# Autodesk Inventor assembly: Assembly-jig
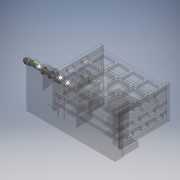
[picture p0: Inventor's stored thumbnail of the model, 180x180]
Saved by Autodesk Inventor 2018 (Build 220112000, 112)
## iProperties
Created: 2017-11-08
Part Number: Assembly-jig
Document SubType Name: Assembly
Designer: xl0
Author: xl0
## Documents named in this file (7)
- E:\Alex\koi\Cuvette-rack\Parts\Assembly-jig\Assembly-jig.iam
- E:\Alex\koi\Cuvette-rack\Parts\Cuvette-rack.iam
- E:\Alex\koi\Cuvette-rack\Parts\Assembly-jig\Assembly-jig-base.ipt
- E:\Alex\koi\Cuvette-rack\Parts\Assembly-jig\Assembly-jig\Design Accelerator\Compress Spring3.iam
- C:\Users\xl0\Documents\Inventor\Content Center Files\R2018\en-US\ANSI B18.2.4.2M\ANSI B18.2.4.2M - M3x0.5 - 5.5.ipt
- C:\Users\xl0\Documents\Inventor\Content Center Files\R2018\en-US\ANSI B18.22 M\ANSI B18.22M - 3 N.ipt
- C:\Users\xl0\Documents\Inventor\Content Center Files\R2018\en-US\SS-ISO 4762\ISO 4762 - M4 x 40SS-ISO.ipt
## Components (8 placed, 6 different names)
1. Cuvette-rack:1 [sub-assembly] — Flush:1, Flush:4
2. Assembly-jig-base:1 — Flush:1, Flush:4, Mate:1, Mate:8, Mate:9
3. SS ISO 4762 M4 x 40:1 — Mate:1, Mate:2, Flush:5, Mate:3, Mate:4, Mate:6, Mate:7, Flush:6
4. Compress Spring:2 [sub-assembly] — Mate:2, Flush:5
5. ANSI B18.2.4.2M M3x0.5:1 — Mate:3, Mate:5
6. ANSI B18.2.4.2M M3x0.5:2 — Mate:4, Mate:5, Flush:6
7. Plain Washer (Metric) 3 N:1 — Mate:7, Mate:9
8. Plain Washer (Metric) 3 N:2 — Mate:6, Mate:8
## Relationships (13: Mate 9, Flush 4)
- Flush:1: Cuvette-rack:1 ↔ Assembly-jig-base:1
- Flush:4 (2 mm): Cuvette-rack:1 ↔ Assembly-jig-base:1
- Mate:1: Assembly-jig-base:1 ↔ SS ISO 4762 M4 x 40:1
- Mate:2: SS ISO 4762 M4 x 40:1 ↔ Compress Spring:2
- Flush:5: SS ISO 4762 M4 x 40:1 ↔ Compress Spring:2
- Mate:3: SS ISO 4762 M4 x 40:1 ↔ ANSI B18.2.4.2M M3x0.5:1
- Mate:4: SS ISO 4762 M4 x 40:1 ↔ ANSI B18.2.4.2M M3x0.5:2
- Mate:5: ANSI B18.2.4.2M M3x0.5:1 ↔ ANSI B18.2.4.2M M3x0.5:2
- Mate:6: SS ISO 4762 M4 x 40:1 ↔ Plain Washer (Metric) 3 N:2
- Mate:7: SS ISO 4762 M4 x 40:1 ↔ Plain Washer (Metric) 3 N:1
- Mate:8: Assembly-jig-base:1 ↔ Plain Washer (Metric) 3 N:2
- Mate:9: Assembly-jig-base:1 ↔ Plain Washer (Metric) 3 N:1
- Flush:6 (-2 mm): SS ISO 4762 M4 x 40:1 ↔ ANSI B18.2.4.2M M3x0.5:2
